# Autodesk Inventor assembly: aerospike assembly
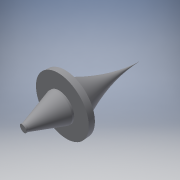
[picture p0: Inventor's stored thumbnail of the model, 180x180]
Saved by Autodesk Inventor 2017 (Build 210142000, 142)
## iProperties
Created: 2016-10-16
Part Number: aerospike assembly
Document SubType Name: Assembly
Designer: Will
Author: Will
## Documents named in this file (3)
- C:\Users\lieub\Desktop\Propulsion\Projects\Aerospike_Trade_Study\aerospike assembly.iam
- C:\Users\lieub\Desktop\Propulsion\Projects\Aerospike_Trade_Study\Spike tip.ipt
- C:\Users\lieub\Desktop\Propulsion\Projects\Aerospike_Trade_Study\Aerospike base.ipt
## Components (2 placed, 2 different names)
1. Spike tip:1 — Insert:1
2. Aerospike base:1 — Insert:1
## Relationships (1: Insert 1)
- Insert:1: Spike tip:1 ↔ Aerospike base:1
